# Autodesk Inventor assembly: Bearing Sled
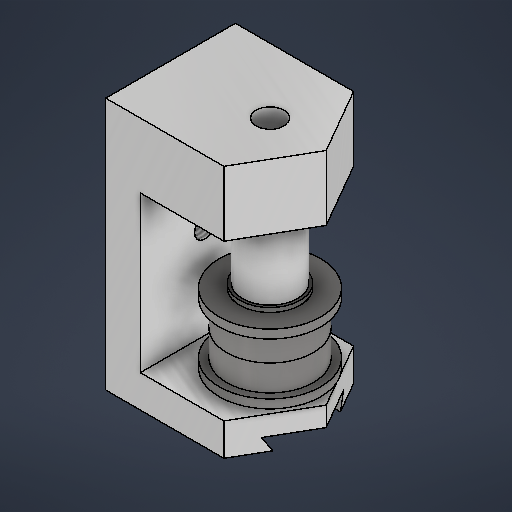
[picture p0: Inventor's stored thumbnail of the model, 512x512]
Saved by Autodesk Inventor 2026 (Build 300175050, 175E)
## iProperties
Created: 2025-05-28
Part Number: Bearing Sled
Document SubType Name: Assembly
Designer: Joshua Eah
Author: Joshua Eah
## Documents named in this file (4)
- C:\Users\Joshua Eah\Documents\GitHub\Voron-0\CAD\Tulip - Machined Parts\Idlers\Bearing Sled.iam
- C:\Users\Joshua Eah\Documents\GitHub\Voron-0\CAD\Tulip - Machined Parts\Idlers\Bearing Sled Single.ipt
- C:\Users\Joshua Eah\Documents\GitHub\Voron-0\CAD\Master Assembly\Hardware\F623 Stack.iam
- C:\Users\Joshua Eah\Documents\GitHub\Voron-0\CAD\Machined Parts\Spacers\Spacer.ipt
## Components (3 placed, 3 different names)
1. Bearing Sled Single:1 — Insert:3
2. F623 Stack:1 [sub-assembly] — Insert:2
3. Spacer:1 — Insert:2, Insert:3
## Relationships (2: Insert 2)
- Insert:2: F623 Stack:1 ↔ Spacer:1
- Insert:3: Bearing Sled Single:1 ↔ Spacer:1
